# Autodesk Inventor assembly: New_hinge_assembly
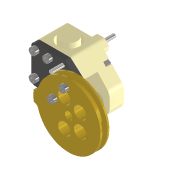
[picture p0: Inventor's stored thumbnail of the model, 180x180]
Saved by Autodesk Inventor 2022 (Build 260153000, 153)
## iProperties
Created: 2022-07-14
Part Number: New_hinge_assembly
Document SubType Name: Assembly
Designer: dell
Mass: 13.3107 g
Surface Area: 105.527 cm^2
Volume: 13.3107 cm^3
Density: 1 g/cm^3
Author: dell
## Documents named in this file (8)
- D:\xxxx\Uni\Part IV\MECHENG_700\Part_IV_project_CAD\Bird_skeleton_prototypes\Wing_drone_V1\Bird_wing_V2\New_hinge_assembly.iam
- D:\xxxx\Uni\Part IV\MECHENG_700\Part_IV_project_CAD\Bird_skeleton_prototypes\Wing_drone_V1\Bird_wing_V2\New_hinge.ipt
- D:\xxxx\Uni\Part IV\MECHENG_700\Part_IV_project_CAD\Bird_skeleton_prototypes\Wing_drone_V1\Bird_wing_V2\New_hinge_plate.ipt
- D:\xxxx\Uni\Part IV\MECHENG_700\Part_IV_project_CAD\Bird_skeleton_prototypes\Wing_drone_V1\Bird_wing_V2\New_coupling_pulley_p1.ipt
- D:\xxxx\Uni\Part IV\MECHENG_700\Part_IV_project_CAD\Bird_skeleton_prototypes\Wing_drone_V1\Bird_wing_V2\Hinge_bearing.ipt
- D:\xxxx\Uni\Part IV\MECHENG_700\Part_IV_project_CAD\Bird_skeleton_prototypes\Wing_drone_V1\Bird_wing_V2\M2_nut.ipt
- D:\xxxx\Uni\Part IV\MECHENG_700\Part_IV_project_CAD\Bird_skeleton_prototypes\Wing_drone_V1\Bird_wing_V2\M2_bolt.ipt
- D:\xxxx\Uni\Part IV\MECHENG_700\Part_IV_project_CAD\Bird_skeleton_prototypes\Wing_drone_V1\Bird_wing_V2\M2_pin.ipt
## Components (19 placed, 7 different names)
1. New_hinge:1 — Mate:1, Mate:2, Mate:6, Mate:7, Mate:8, Mate:15, Mate:16, Mate:19, Mate:20, Mate:21, Mate:22, Mate:23, Mate:24, Mate:25, Mate:26, Mate:27, Mate:28
2. New_hinge:2 — Mate:1, Mate:2, Mate:3, Mate:4, Mate:5
3. New_hinge_plate:3 — Mate:3, Mate:4, Mate:5, Mate:12, Mate:13, Mate:14
4. New_hinge_plate:4 — Mate:6, Mate:7, Mate:8, Mate:9, Mate:10, Mate:11, Mate:17, Mate:29, Mate:30, Mate:31, Mate:32, Mate:37, Mate:38, Mate:39, Flush:1
5. New_coupling_pulley_p1:1 — Mate:9, Mate:10, Mate:11, Mate:18, Mate:33, Mate:34, Mate:35, Mate:36
6. New_coupling_pulley_p1:2 — Mate:12, Mate:13, Mate:14
7. Hinge_bearing:1 — Mate:15, Mate:19
8. Hinge_bearing:2 — Mate:16, Mate:20
9. Hinge_bearing:3 — Mate:17, Mate:18
10. M2_nut:1 — Mate:22, Mate:26
11. M2_nut:2 — Mate:24, Mate:25
12. M2_nut:3 — Mate:23, Mate:28
13. M2_nut:4 — Mate:21, Mate:27
14. M2_bolt:1 — Mate:31, Mate:32
15. M2_bolt:2 — Mate:33, Mate:34
16. M2_bolt:3 — Mate:35, Mate:36
17. M2_bolt:4 — Mate:29, Mate:30
18. M2_bolt:5 — Mate:37, Mate:38
19. M2_pin:1 — Mate:39, Flush:1
## Relationships (40: Mate 39, Flush 1)
- Mate:1: New_hinge:1 ↔ New_hinge:2
- Mate:2: New_hinge:1 ↔ New_hinge:2
- Mate:3: New_hinge:2 ↔ New_hinge_plate:3
- Mate:4: New_hinge:2 ↔ New_hinge_plate:3
- Mate:5: New_hinge:2 ↔ New_hinge_plate:3
- Mate:6: New_hinge:1 ↔ New_hinge_plate:4
- Mate:7: New_hinge:1 ↔ New_hinge_plate:4
- Mate:8: New_hinge:1 ↔ New_hinge_plate:4
- Mate:9: New_hinge_plate:4 ↔ New_coupling_pulley_p1:1
- Mate:10: New_hinge_plate:4 ↔ New_coupling_pulley_p1:1
- Mate:11: New_hinge_plate:4 ↔ New_coupling_pulley_p1:1
- Mate:12: New_hinge_plate:3 ↔ New_coupling_pulley_p1:2
- Mate:13: New_hinge_plate:3 ↔ New_coupling_pulley_p1:2
- Mate:14: New_hinge_plate:3 ↔ New_coupling_pulley_p1:2
- Mate:15: New_hinge:1 ↔ Hinge_bearing:1
- Mate:16: New_hinge:1 ↔ Hinge_bearing:2
- Mate:17: New_hinge_plate:4 ↔ Hinge_bearing:3
- Mate:18: New_coupling_pulley_p1:1 ↔ Hinge_bearing:3
- Mate:19: New_hinge:1 ↔ Hinge_bearing:1
- Mate:20: New_hinge:1 ↔ Hinge_bearing:2
- Mate:21: New_hinge:1 ↔ M2_nut:4
- Mate:22: New_hinge:1 ↔ M2_nut:1
- Mate:23: New_hinge:1 ↔ M2_nut:3
- Mate:24: New_hinge:1 ↔ M2_nut:2
- Mate:25: New_hinge:1 ↔ M2_nut:2
- Mate:26: New_hinge:1 ↔ M2_nut:1
- Mate:27: New_hinge:1 ↔ M2_nut:4
- Mate:28: New_hinge:1 ↔ M2_nut:3
- Mate:29: New_hinge_plate:4 ↔ M2_bolt:4
- Mate:30: New_hinge_plate:4 ↔ M2_bolt:4
- Mate:31: New_hinge_plate:4 ↔ M2_bolt:1
- Mate:32: New_hinge_plate:4 ↔ M2_bolt:1
- Mate:33: New_coupling_pulley_p1:1 ↔ M2_bolt:2
- Mate:34: New_coupling_pulley_p1:1 ↔ M2_bolt:2
- Mate:35: New_coupling_pulley_p1:1 ↔ M2_bolt:3
- Mate:36: New_coupling_pulley_p1:1 ↔ M2_bolt:3
- Mate:37: New_hinge_plate:4 ↔ M2_bolt:5
- Mate:38: New_hinge_plate:4 ↔ M2_bolt:5
- Mate:39: New_hinge_plate:4 ↔ M2_pin:1
- Flush:1 (-6.8 mm): New_hinge_plate:4 ↔ M2_pin:1
